# Autodesk Inventor assembly: Kontaktpins_Gerade
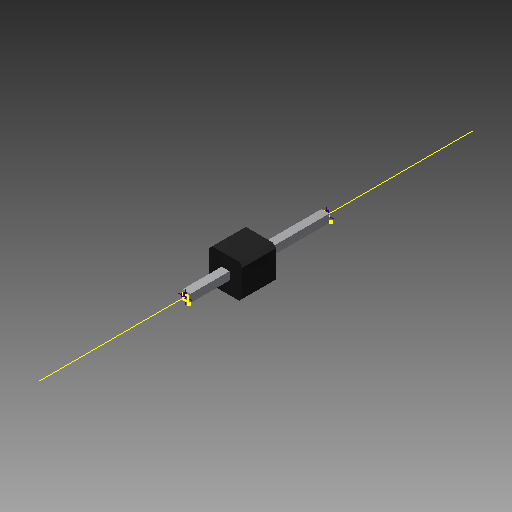
[picture p0: Inventor's stored thumbnail of the model, 512x512]
Saved by Autodesk Inventor 2019 (Build 230136000, 136)
## iProperties
Created: 2019-03-11
Part Number: Kontaktpins_Gerade
Material: Generisch
Document SubType Name: Assembly
Designer: manue
Author: manue
## Documents named in this file (3)
- E:\Benutzer\manue\Nextcloud\Unterlagen\Studium\OTH AMBERG\Industrie 4.0\Semester 4\Projektmanagement & agile Projektmethoden\Projekt Sensornetzwerk\Sensorknoten\ModellV1.1\MQ135\Kontaktpins_Gerade.iam
- E:\Benutzer\manue\Nextcloud\Unterlagen\Studium\OTH AMBERG\Industrie 4.0\Semester 4\Projektmanagement & agile Projektmethoden\Projekt Sensornetzwerk\Sensorknoten\ModellV1.1\MQ135\Pins.ipt
- E:\Benutzer\manue\Nextcloud\Unterlagen\Studium\OTH AMBERG\Industrie 4.0\Semester 4\Projektmanagement & agile Projektmethoden\Projekt Sensornetzwerk\Sensorknoten\ModellV1.1\MQ135\Kontakthalter.ipt
## Components (2 placed, 2 different names)
1. Pins:1 — Fluchtend:1
2. Kontakthalter:1 — Fluchtend:2, Fluchtend:3
## Relationships (3: Flush 3)
- Fluchtend:1 [Flush] (-5.6 mm): Pins:1
- Fluchtend:2 [Flush]: Kontakthalter:1
- Fluchtend:3 [Flush]: Kontakthalter:1
